# Autodesk Inventor assembly: US com sup
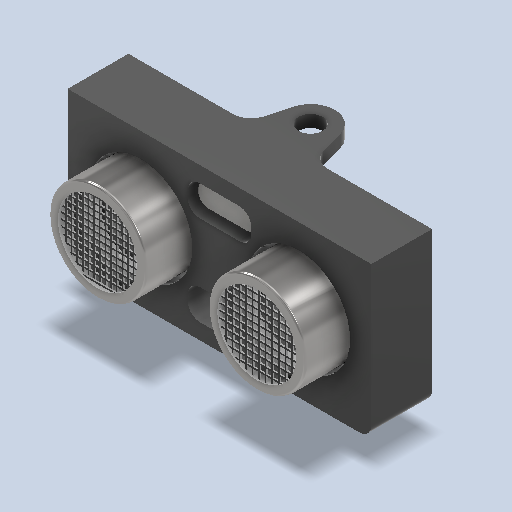
[picture p0: Inventor's stored thumbnail of the model, 512x512]
Saved by Autodesk Inventor 2025.1 (Build 291241000, 241)
## iProperties
Created: 2024-09-06
Part Number: US com sup
Document SubType Name: Assembly
Designer: Célio
Author: Célio
## Documents named in this file (3)
- C:\Users\Aluno\Downloads\carrinho\partes\US com sup.iam
- C:\Users\Aluno\Downloads\carrinho\partes\ultrasonic-sensor-hc-sr04-1.snapshot.1\HC-SR04-UltrasonicSensor v7 v2.ipt
- C:\Users\Aluno\Downloads\carrinho\partes\suporte ultrasom.ipt
## Components (2 placed, 2 different names)
1. HC-SR04-UltrasonicSensor v7 v2:1 — Alinhado:1
2. suporte ultrasom:1 — Alinhado:1
## Relationships (1: Flush 1)
- Alinhado:1 [Flush]: HC-SR04-UltrasonicSensor v7 v2:1 ↔ suporte ultrasom:1
